# Autodesk Inventor assembly: EOD_D1_v2.0
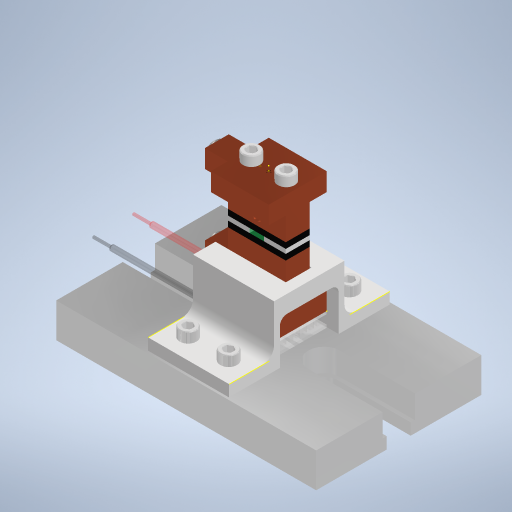
[picture p0: Inventor's stored thumbnail of the model, 512x512]
Saved by Autodesk Inventor 2024.2 (Build 282272000, 272)
## iProperties
Created: 2023-03-15
Part Number: EOD_D1_v2.0
Document SubType Name: Assembly
Designer: warke
Author: warke
## Documents named in this file (12)
- G:\Shared drives\Kerlin lab shared\Users\ChrisW\EOD\Builds\device1_032024\EOD_D1_v2.0.iam
- G:\Shared drives\Kerlin lab shared\Users\ChrisW\EOD\Builds\pckngo\ledgerEOD_v1.0\bottomblock_Cu_LEOD.ipt
- G:\Shared drives\Kerlin lab shared\Users\ChrisW\EOD\Builds\pckngo\toplitEOD_v1.0\TEC3-2.5-Solidworks (1).ipt
- G:\Shared drives\Kerlin lab shared\Users\ChrisW\EOD\Builds\pckngo\ledgerEOD_v1.0\electrode_Cu_LEOD.ipt
- G:\Shared drives\Kerlin lab shared\Users\ChrisW\EOD\Builds\pckngo\ledgerEOD_v1.0\peltierclip_LEOD.ipt
- G:\Shared drives\Kerlin lab shared\Users\ChrisW\EOD\Builds\pckngo\ledgerEOD_v1.0\KTN_Chip_6p6mm_4mm_1p2mm_WithElectrodes.ipt
- G:\Shared drives\Kerlin lab shared\Users\ChrisW\EOD\Builds\pckngo\ledgerEOD_v1.0\graphite_LEOD.ipt
- G:\Shared drives\Kerlin lab shared\Users\ChrisW\EOD\Builds\pckngo\ledgerEOD_v1.0\92949A105_18-8 Stainless Steel Button Head Hex Drive Screw.ipt
- G:\Shared drives\Kerlin lab shared\Users\ChrisW\EOD\Builds\pckngo\toplitEOD_v1.0\92196A107_18-8 Stainless Steel Socket Head Screw.ipt
- G:\Shared drives\Kerlin lab shared\Users\ChrisW\EOD\Builds\pckngo\ledgerEOD_v1.0\spacer_AlN_LEOD.ipt
- G:\Shared drives\Kerlin lab shared\Users\ChrisW\EOD\Builds\pckngo\ledgerEOD_v1.0\base_Al_LEOD.ipt
- G:\Shared drives\Kerlin lab shared\Users\ChrisW\EOD\Builds\ledger_EOD_03223\95868A117_Nylon Socket Head Screws.ipt
## Components (18 placed, 11 different names)
1. TEC3-2.5-Solidworks (1):1 — Mate:25
2. bottomblock_Cu_LEOD:2 — Mate:3
3. electrode_Cu_LEOD:1 — Mate:3, Mate:5, Mate:22
4. electrode_Cu_LEOD:2 — Mate:9, Mate:20, Mate:21, Mate:26, Mate:27
5. peltierclip_LEOD:1 — Mate:16, Mate:17, Mate:18, Mate:19
6. graphite_LEOD:1 — Mate:8, Mate:9
7. graphite_LEOD:2 — Mate:5, Mate:6, Mate:23, Mate:24
8. KTN_Chip_6p6mm_4mm_1p2mm_WithElectrodes:1 — Mate:6, Mate:8
9. 92949A105_18-8 Stainless Steel Button Head Hex Drive Screw:1 — Mate:22
10. 92949A105_18-8 Stainless Steel Button Head Hex Drive Screw:2 — Mate:20, Mate:21
11. 92196A107_18-8 Stainless Steel Socket Head Screw:1 — Mate:16
12. 92196A107_18-8 Stainless Steel Socket Head Screw:2 — Mate:18
13. 92196A107_18-8 Stainless Steel Socket Head Screw:3 — Mate:17
14. 92196A107_18-8 Stainless Steel Socket Head Screw:4 — Mate:19
15. spacer_AlN_LEOD:1 — Mate:23, Mate:24
16. base_Al_LEOD:1 — Mate:25
17. 95868A117_Nylon Socket Head Screws:1 — Mate:26
18. 95868A117_Nylon Socket Head Screws:2 — Mate:27
## Relationships (17: Mate 17)
- Mate:3: bottomblock_Cu_LEOD:2 ↔ electrode_Cu_LEOD:1
- Mate:5: electrode_Cu_LEOD:1 ↔ graphite_LEOD:2
- Mate:6: graphite_LEOD:2 ↔ KTN_Chip_6p6mm_4mm_1p2mm_WithElectrodes:1
- Mate:8: graphite_LEOD:1 ↔ KTN_Chip_6p6mm_4mm_1p2mm_WithElectrodes:1
- Mate:9: electrode_Cu_LEOD:2 ↔ graphite_LEOD:1
- Mate:16: peltierclip_LEOD:1 ↔ 92196A107_18-8 Stainless Steel Socket Head Screw:1
- Mate:17: peltierclip_LEOD:1 ↔ 92196A107_18-8 Stainless Steel Socket Head Screw:3
- Mate:18: peltierclip_LEOD:1 ↔ 92196A107_18-8 Stainless Steel Socket Head Screw:2
- Mate:19: peltierclip_LEOD:1 ↔ 92196A107_18-8 Stainless Steel Socket Head Screw:4
- Mate:20: electrode_Cu_LEOD:2 ↔ 92949A105_18-8 Stainless Steel Button Head Hex Drive Screw:2
- Mate:21: electrode_Cu_LEOD:2 ↔ 92949A105_18-8 Stainless Steel Button Head Hex Drive Screw:2
- Mate:22: electrode_Cu_LEOD:1 ↔ 92949A105_18-8 Stainless Steel Button Head Hex Drive Screw:1
- Mate:23: graphite_LEOD:2 ↔ spacer_AlN_LEOD:1
- Mate:24: graphite_LEOD:2 ↔ spacer_AlN_LEOD:1
- Mate:25: TEC3-2.5-Solidworks (1):1 ↔ base_Al_LEOD:1
- Mate:26: electrode_Cu_LEOD:2 ↔ 95868A117_Nylon Socket Head Screws:1
- Mate:27: electrode_Cu_LEOD:2 ↔ 95868A117_Nylon Socket Head Screws:2
